# Autodesk Inventor assembly: Controller Box
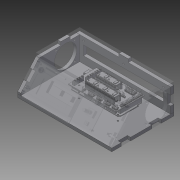
[picture p0: Inventor's stored thumbnail of the model, 180x180]
Saved by Autodesk Inventor 2014 (Build 180170000, 170)
## iProperties
Created: 2014-11-10
Part Number: Controller Box
Document SubType Name: Assembly
Designer: ThatOtherGuy
Author: ThatOtherGuy
## Documents named in this file (8)
- C:\Users\ThatOtherGuy\Documents\Inventor\KosselCNC1515\Mounts\Controller Box.iam
- C:\Users\ThatOtherGuy\Documents\Inventor\KosselCNC1515\Mounts\Controller_Base.ipt
- C:\Users\ThatOtherGuy\Documents\Inventor\KosselCNC1515\Mounts\Controller_Side_A.ipt
- C:\Users\ThatOtherGuy\Documents\Inventor\KosselCNC1515\Mounts\Controller_Back.ipt
- C:\Users\ThatOtherGuy\Documents\Inventor\KosselCNC1515\Mounts\Controller_Front.ipt
- C:\Users\ThatOtherGuy\Documents\Inventor\KosselCNC1515\Mounts\RepRapDiscount-SmartController\RepRapDiscount_SmartController.ipt
- C:\Users\ThatOtherGuy\Documents\Inventor\KosselCNC1515\Mounts\Controller_Top.ipt
- C:\Users\ThatOtherGuy\Documents\Inventor\KosselCNC1515\Electronics\3DPrinter.iam
## Components (8 placed, 7 different names)
1. Controller_Base:1 — Mate:1, Mate:2, Mate:3, Mate:4, Mate:5, Mate:6, Mate:13, Mate:14, Mate:15, Insert:1, Insert:2
2. Controller_Side_A:1 — Mate:1, Mate:2, Mate:3, Mate:7, Mate:8, Mate:9, Mate:16, Mate:17
3. Controller_Back:1 — Mate:4, Mate:5, Mate:6, Mate:18
4. Controller_Front:1 — Mate:7, Mate:8, Mate:9, Mate:10, Mate:11, Mate:12
5. RepRapDiscount_SmartController:1 — Mate:10, Mate:11, Mate:12
6. Controller_Side_A:2 — Mate:13, Mate:14, Mate:15
7. Controller_Top:1 — Mate:16, Mate:17, Mate:18
8. 3DPrinter:1 [sub-assembly] — Insert:1, Insert:2
## Relationships (20: Mate 18, Insert 2)
- Mate:1: Controller_Base:1 ↔ Controller_Side_A:1
- Mate:2: Controller_Base:1 ↔ Controller_Side_A:1
- Mate:3: Controller_Base:1 ↔ Controller_Side_A:1
- Mate:4: Controller_Base:1 ↔ Controller_Back:1
- Mate:5: Controller_Base:1 ↔ Controller_Back:1
- Mate:6: Controller_Base:1 ↔ Controller_Back:1
- Mate:7: Controller_Side_A:1 ↔ Controller_Front:1
- Mate:8: Controller_Side_A:1 ↔ Controller_Front:1
- Mate:9: Controller_Side_A:1 ↔ Controller_Front:1
- Mate:10: Controller_Front:1 ↔ RepRapDiscount_SmartController:1
- Mate:11: Controller_Front:1 ↔ RepRapDiscount_SmartController:1
- Mate:12 (2.5 mm): Controller_Front:1 ↔ RepRapDiscount_SmartController:1
- Mate:13: Controller_Base:1 ↔ Controller_Side_A:2
- Mate:14: Controller_Base:1 ↔ Controller_Side_A:2
- Mate:15: Controller_Base:1 ↔ Controller_Side_A:2
- Mate:16: Controller_Side_A:1 ↔ Controller_Top:1
- Mate:17: Controller_Side_A:1 ↔ Controller_Top:1
- Mate:18: Controller_Back:1 ↔ Controller_Top:1
- Insert:1 (10 mm): Controller_Base:1 ↔ 3DPrinter:1
- Insert:2 (10 mm): Controller_Base:1 ↔ 3DPrinter:1
